# Autodesk Inventor assembly: Assembly
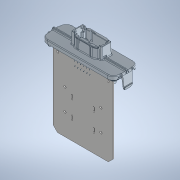
[picture p0: Inventor's stored thumbnail of the model, 180x180]
Saved by Autodesk Inventor 2021 (Build 250183000, 183)
## iProperties
Created: 2020-09-13
Part Number: Assembly
Document SubType Name: Assembly
Designer: Viktor
Author: Viktor
## Documents named in this file (5)
- C:\Users\Viktor\Documents\GitHub\WaveRunner-CCU\RCU\hw\CAD\Assembly.iam
- C:\Users\Viktor\Documents\GitHub\WaveRunner-CCU\RCU\hw\CAD\c-eec-325x4a-e016-99-3d.ipt
- C:\Users\Viktor\Documents\GitHub\WaveRunner-CCU\RCU\hw\CAD\FrSky_RX8R.ipt
- C:\Users\Viktor\Documents\GitHub\WaveRunner-CCU\RCU\hw\CAD\PCB.ipt
- C:\Users\Viktor\Documents\GitHub\WaveRunner-CCU\RCU\hw\CAD\c-dtm13-12pa-r008-c-3d.ipt
## Components (4 placed, 4 different names)
1. c-eec-325x4a-e016-99-3d:1 — Rigid:2
2. FrSky_RX8R:1
3. PCB:1 — Rigid:1
4. c-dtm13-12pa-r008-c-3d:2 — Rigid:1, Rigid:2
## Relationships (2: WeldJoint 2)
- Rigid:1 [WeldJoint] (-0.381 mm): PCB:1 ↔ c-dtm13-12pa-r008-c-3d:2
- Rigid:2 [WeldJoint]: c-eec-325x4a-e016-99-3d:1 ↔ c-dtm13-12pa-r008-c-3d:2
